# Autodesk Inventor assembly: Ankle_MIR
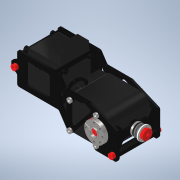
[picture p0: Inventor's stored thumbnail of the model, 180x180]
Saved by Autodesk Inventor 2022.3 (Build 263350000, 350)
## iProperties
Created: 2022-06-04
Part Number: Ankle_MIR
Document SubType Name: Assembly
Designer: Masato Kubotera
Author: Masato Kubotera
## Documents named in this file (19)
- C:\Users\Masato\Documents\Inventor\CIT Brains\SUSTAINA-OP - mod\LowerBody\Ankle\Ankle_MIR.iam
- C:\Users\Masato\Documents\Inventor\CIT Brains\SUSTAINA-OP - mod\LowerBody\Ankle\Ankle_side_frame.ipt
- C:\Users\Masato\Documents\Inventor\CIT Brains\SUSTAINA-OP - mod\LowerBody\Ankle\Ankle_front_frame.ipt
- C:\Users\Masato\Documents\Inventor\CIT Brains\SUSTAINA-OP - mod\LowerBody\Ankle\Ankle_back_frame.ipt
- C:\Users\Masato\Documents\Inventor\CIT Brains\SUSTAINA-OP - mod\ReadyMade\KONDO\B3M-SC-1170-A_with_ClampHorn_AND_FreeHorn.iam
- C:\Users\Masato\Documents\Inventor\CIT Brains\SUSTAINA-OP - mod\ReadyMade\KONDO\B3M-SC-1040-A_with_ClampHorn.iam
- C:\Users\Masato\Documents\Inventor\CIT Brains\SUSTAINA-OP - mod\ReadyMade\Spacer\ABLSBF6-39.5-M3-N3.ipt
- C:\Users\Masato\Documents\Inventor\CIT Brains\SUSTAINA-OP - mod\ReadyMade\InsertNut\S4-05-3W.ipt
- C:\Users\Masato\Documents\Inventor\CIT Brains\SUSTAINA-OP - mod\ReadyMade\Washer\CC-0612-15B.ipt
- C:\Users\Masato\Documents\Inventor\CIT Brains\SUSTAINA-OP - mod\ReadyMade\Bush\80F-0603.ipt
- C:\Users\Masato\Documents\Inventor\CIT Brains\SUSTAINA-OP - mod\ReadyMade\Washer\TT-0814-10.ipt
- C:\Users\Masato\Documents\Inventor\CIT Brains\SUSTAINA-OP - mod\ReadyMade\Washer\UUW-0614-03H.ipt
- C:\Users\Masato\Documents\Inventor\CIT Brains\SUSTAINA-OP - mod\ReadyMade\Screw\UC-0306.ipt
- C:\Users\Masato\Documents\Inventor\CIT Brains\SUSTAINA-OP - mod\ReadyMade\Screw\FC-2615EB.ipt
- C:\Users\Masato\Documents\Inventor\CIT Brains\SUSTAINA-OP - mod\ReadyMade\Screw\FC-2620EB.ipt
- C:\Users\Masato\Documents\Inventor\CIT Brains\SUSTAINA-OP - mod\ReadyMade\Screw\LowHead_M2_6-15.ipt
- C:\Users\Masato\Documents\Inventor\CIT Brains\SUSTAINA-OP - mod\ReadyMade\Screw\LowHead_M2_6-20.ipt
- C:\Users\Masato\Documents\Inventor\CIT Brains\SUSTAINA-OP - mod\ReadyMade\Screw\DBTS4-7-5-DHC.ipt
- C:\Users\Masato\Documents\Inventor\CIT Brains\SUSTAINA-OP - mod\ReadyMade\Washer\UUW-0412-20H.ipt
## Components (34 placed, 18 different names)
1. Ankle_side_frame:1 — フラッシュ:4, メイト:3, メイト:2, フラッシュ:5, メイト:5, メイト:4, 挿入:4, 挿入:3, 挿入:2, 挿入:1, 角度:1, 挿入:9, 角度:2, 挿入:11, 挿入:26, 挿入:28, 挿入:44, 挿入:45, 挿入:46, 挿入:47
2. Ankle_side_frame:2 — 挿入:12, 挿入:10, 挿入:8, 挿入:7, 挿入:6, 挿入:5, 挿入:27, 挿入:29, 挿入:48, 挿入:49, 挿入:50, 挿入:51
3. Ankle_front_frame:1 — フラッシュ:4, メイト:3, メイト:2, メイト:1, 挿入:19, Insert:53
4. Ankle_back_frame:1 — 挿入:18, 挿入:17, 挿入:16, 挿入:15, 挿入:40, 挿入:41, 挿入:42, 挿入:43
5. Ankle_back_frame:2 — フラッシュ:5, メイト:5, メイト:4, 挿入:14, 挿入:13, 挿入:38, 挿入:39
6. B3M-SC-1170-A_with_ClampHorn_AND_FreeHorn:1 [sub-assembly] — 挿入:4, 挿入:3, 挿入:2, 挿入:1, フラッシュ:3, フラッシュ:2, フラッシュ:1, 挿入:8, 挿入:7, 挿入:6, 挿入:5
7. B3M-SC-1040-A_with_ClampHorn:1 [sub-assembly] — 挿入:18, 挿入:17, 挿入:16, 挿入:15, 挿入:14, 挿入:13
8. ABLSBF6-39.5-M3-N3:1 — 角度:1, 挿入:9, 挿入:10
9. ABLSBF6-39.5-M3-N3:2 — 角度:2, 挿入:11, 挿入:12
10. S4-05-3W:1 — メイト:1, 挿入:19
11. CC-0612-15B:1 — 挿入:22, Insert:54
12. 80F-0603:1 — 挿入:22
13. TT-0814-10:1 — 挿入:25
14. UUW-0614-03H:1 — 挿入:25, Insert:52
15. UC-0306:1 — 挿入:26
16. UC-0306:2 — 挿入:27
17. UC-0306:3 — 挿入:28
18. UC-0306:4 — 挿入:29
19. FC-2620EB:3 — 挿入:38
20. FC-2620EB:4 — 挿入:39
21. FC-2615EB:5 — 挿入:40
22. FC-2615EB:6 — 挿入:41
23. FC-2615EB:7 — 挿入:42
24. FC-2615EB:8 — 挿入:43
25. LowHead_M2_6-15:1 — 挿入:44
26. LowHead_M2_6-15:2 — 挿入:45
27. LowHead_M2_6-15:3 — 挿入:46
28. LowHead_M2_6-15:4 — 挿入:47
29. LowHead_M2_6-20:1 — 挿入:48
30. LowHead_M2_6-20:2 — 挿入:49
31. LowHead_M2_6-20:3 — 挿入:50
32. LowHead_M2_6-20:4 — 挿入:51
33. DBTS4-7-5-DHC:1 — Insert:52, Insert:55
34. UUW-0412-20H:1 — Insert:53, Insert:54, Insert:55
## Relationships (55: Insert 43, Mate 6, Flush 4, Angle 2)
- フラッシュ:4 [Flush]: Ankle_side_frame:1 ↔ Ankle_front_frame:1
- メイト:3 [Mate] (0.025 mm): Ankle_side_frame:1 ↔ Ankle_front_frame:1
- メイト:2 [Mate] (0.025 mm): Ankle_side_frame:1 ↔ Ankle_front_frame:1
- フラッシュ:5 [Flush]: Ankle_side_frame:1 ↔ Ankle_back_frame:2
- メイト:5 [Mate] (0.025 mm): Ankle_side_frame:1 ↔ Ankle_back_frame:2
- メイト:4 [Mate] (0.025 mm): Ankle_side_frame:1 ↔ Ankle_back_frame:2
- 挿入:18 [Insert]: Ankle_back_frame:1 ↔ B3M-SC-1040-A_with_ClampHorn:1
- 挿入:17 [Insert]: Ankle_back_frame:1 ↔ B3M-SC-1040-A_with_ClampHorn:1
- 挿入:16 [Insert]: Ankle_back_frame:1 ↔ B3M-SC-1040-A_with_ClampHorn:1
- 挿入:15 [Insert]: Ankle_back_frame:1 ↔ B3M-SC-1040-A_with_ClampHorn:1
- 挿入:14 [Insert]: Ankle_back_frame:2 ↔ B3M-SC-1040-A_with_ClampHorn:1
- 挿入:13 [Insert]: Ankle_back_frame:2 ↔ B3M-SC-1040-A_with_ClampHorn:1
- 挿入:4 [Insert]: Ankle_side_frame:1 ↔ B3M-SC-1170-A_with_ClampHorn_AND_FreeHorn:1
- 挿入:3 [Insert]: Ankle_side_frame:1 ↔ B3M-SC-1170-A_with_ClampHorn_AND_FreeHorn:1
- 挿入:2 [Insert]: Ankle_side_frame:1 ↔ B3M-SC-1170-A_with_ClampHorn_AND_FreeHorn:1
- 挿入:1 [Insert]: Ankle_side_frame:1 ↔ B3M-SC-1170-A_with_ClampHorn_AND_FreeHorn:1
- フラッシュ:3 [Flush]: B3M-SC-1170-A_with_ClampHorn_AND_FreeHorn:1
- フラッシュ:2 [Flush]: B3M-SC-1170-A_with_ClampHorn_AND_FreeHorn:1
- フラッシュ:1 [Mate]: B3M-SC-1170-A_with_ClampHorn_AND_FreeHorn:1
- 角度:1 [Angle] (0 deg): Ankle_side_frame:1 ↔ ABLSBF6-39.5-M3-N3:1
- 挿入:9 [Insert]: Ankle_side_frame:1 ↔ ABLSBF6-39.5-M3-N3:1
- 角度:2 [Angle] (0 deg): Ankle_side_frame:1 ↔ ABLSBF6-39.5-M3-N3:2
- 挿入:11 [Insert]: Ankle_side_frame:1 ↔ ABLSBF6-39.5-M3-N3:2
- 挿入:12 [Insert]: Ankle_side_frame:2 ↔ ABLSBF6-39.5-M3-N3:2
- 挿入:10 [Insert]: Ankle_side_frame:2 ↔ ABLSBF6-39.5-M3-N3:1
- 挿入:8 [Insert]: Ankle_side_frame:2 ↔ B3M-SC-1170-A_with_ClampHorn_AND_FreeHorn:1
- 挿入:7 [Insert]: Ankle_side_frame:2 ↔ B3M-SC-1170-A_with_ClampHorn_AND_FreeHorn:1
- 挿入:6 [Insert]: Ankle_side_frame:2 ↔ B3M-SC-1170-A_with_ClampHorn_AND_FreeHorn:1
- 挿入:5 [Insert]: Ankle_side_frame:2 ↔ B3M-SC-1170-A_with_ClampHorn_AND_FreeHorn:1
- メイト:1 [Mate]: Ankle_front_frame:1 ↔ S4-05-3W:1
- 挿入:19 [Insert]: Ankle_front_frame:1 ↔ S4-05-3W:1
- 挿入:22 [Insert]: CC-0612-15B:1 ↔ 80F-0603:1
- 挿入:26 [Insert]: Ankle_side_frame:1 ↔ UC-0306:1
- 挿入:27 [Insert]: Ankle_side_frame:2 ↔ UC-0306:2
- 挿入:28 [Insert]: Ankle_side_frame:1 ↔ UC-0306:3
- 挿入:29 [Insert]: Ankle_side_frame:2 ↔ UC-0306:4
- 挿入:38 [Insert]: Ankle_back_frame:2 ↔ FC-2620EB:3
- 挿入:39 [Insert]: Ankle_back_frame:2 ↔ FC-2620EB:4
- 挿入:40 [Insert]: Ankle_back_frame:1 ↔ FC-2615EB:5
- 挿入:41 [Insert]: Ankle_back_frame:1 ↔ FC-2615EB:6
- 挿入:42 [Insert]: Ankle_back_frame:1 ↔ FC-2615EB:7
- 挿入:43 [Insert]: Ankle_back_frame:1 ↔ FC-2615EB:8
- 挿入:25 [Insert]: TT-0814-10:1 ↔ UUW-0614-03H:1
- 挿入:44 [Insert]: Ankle_side_frame:1 ↔ LowHead_M2_6-15:1
- 挿入:45 [Insert]: Ankle_side_frame:1 ↔ LowHead_M2_6-15:2
- 挿入:46 [Insert]: Ankle_side_frame:1 ↔ LowHead_M2_6-15:3
- 挿入:47 [Insert]: Ankle_side_frame:1 ↔ LowHead_M2_6-15:4
- 挿入:48 [Insert]: Ankle_side_frame:2 ↔ LowHead_M2_6-20:1
- 挿入:49 [Insert]: Ankle_side_frame:2 ↔ LowHead_M2_6-20:2
- 挿入:50 [Insert]: Ankle_side_frame:2 ↔ LowHead_M2_6-20:3
- 挿入:51 [Insert]: Ankle_side_frame:2 ↔ LowHead_M2_6-20:4
- Insert:52: UUW-0614-03H:1 ↔ DBTS4-7-5-DHC:1
- Insert:53: Ankle_front_frame:1 ↔ UUW-0412-20H:1
- Insert:54: CC-0612-15B:1 ↔ UUW-0412-20H:1
- Insert:55: DBTS4-7-5-DHC:1 ↔ UUW-0412-20H:1
